# Autodesk Inventor assembly: 2024-210-Angle-Shootaur
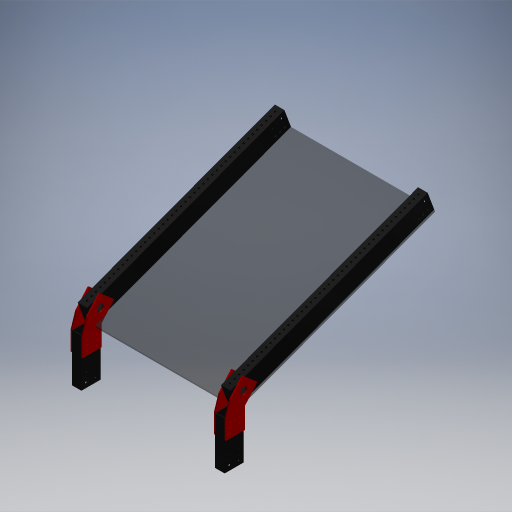
[picture p0: Inventor's stored thumbnail of the model, 512x512]
Saved by Autodesk Inventor 2024.2 (Build 282272000, 272)
## iProperties
Created: 2024-01-23
Part Number: 2024-210-Angle-Shootaur
Document SubType Name: Assembly
Designer: rohan
Author: rohan
## Documents named in this file (5)
- C:\Users\rohan\OneDrive - Hillsborough County Public Schools\Robotics\FIRST-Robotics-Competition\Crescendo\Minotaur-Crescendo-Robot\Structure\Superstructure\Angle-Shootaur\2024-210-Angle-Shootaur.iam
- C:\Users\rohan\OneDrive - Hillsborough County Public Schools\Robotics\FIRST-Robotics-Competition\Crescendo\Minotaur-Crescendo-Robot\Structure\Superstructure\Angle-Shootaur\2024-210-003-Dead-Axle-Gusset.ipt
- C:\Users\rohan\OneDrive - Hillsborough County Public Schools\Robotics\FIRST-Robotics-Competition\Crescendo\Minotaur-Crescendo-Robot\Structure\Superstructure\Angle-Shootaur\2024-210-002-Angle-Beam.ipt
- C:\Users\rohan\OneDrive - Hillsborough County Public Schools\Robotics\FIRST-Robotics-Competition\Crescendo\Minotaur-Crescendo-Robot\Structure\Superstructure\Angle-Shootaur\2024-210-001-Backright-Support.ipt
- C:\Users\rohan\OneDrive - Hillsborough County Public Schools\Robotics\FIRST-Robotics-Competition\Crescendo\Minotaur-Crescendo-Robot\Structure\Superstructure\Polycarbonate-Note-Rest.ipt
## Components (9 placed, 4 different names)
1. 2024-210-003-Dead-Axle-Gusset:1 — Flush:1, Flush:2, Mate:1, Mate:4, Insert:1, Insert:2, Rotational:1
2. 2024-210-003-Dead-Axle-Gusset:2 — Flush:1, Flush:2, Mate:1
3. 2024-210-002-Angle-Beam:1 — Rotational:1, Flush:5, Mate:8, Flush:7, Flush:8
4. 2024-210-001-Backright-Support:1 — Mate:4, Insert:1, Insert:2, Flush:6, Mate:7
5. 2024-210-003-Dead-Axle-Gusset:3
6. 2024-210-003-Dead-Axle-Gusset:4
7. 2024-210-002-Angle-Beam:2 — Flush:5
8. 2024-210-001-Backright-Support:2 — Flush:6, Mate:7
9. Polycarbonate-Note-Rest:1 — Mate:8, Flush:7, Flush:8
## Relationships (20: Flush 8, Mate 6, Insert 4, RevoluteJoint 2)
- Flush:1: 2024-210-003-Dead-Axle-Gusset:1 ↔ 2024-210-003-Dead-Axle-Gusset:2
- Flush:2: 2024-210-003-Dead-Axle-Gusset:1 ↔ 2024-210-003-Dead-Axle-Gusset:2
- Mate:1 (25.4 mm): 2024-210-003-Dead-Axle-Gusset:1 ↔ 2024-210-003-Dead-Axle-Gusset:2
- Mate:4: 2024-210-003-Dead-Axle-Gusset:1 ↔ 2024-210-001-Backright-Support:1
- Insert:1: 2024-210-003-Dead-Axle-Gusset:1 ↔ 2024-210-001-Backright-Support:1
- Insert:2: 2024-210-003-Dead-Axle-Gusset:1 ↔ 2024-210-001-Backright-Support:1
- Rotational:1 [RevoluteJoint] (-3.175 mm): 2024-210-003-Dead-Axle-Gusset:1 ↔ 2024-210-002-Angle-Beam:1
- [Flush]: 2024-210-003-Dead-Axle-Gusset:3 ↔ 2024-210-003-Dead-Axle-Gusset:4
- [Flush]: 2024-210-003-Dead-Axle-Gusset:3 ↔ 2024-210-003-Dead-Axle-Gusset:4
- [Mate] (25.4 mm): 2024-210-003-Dead-Axle-Gusset:3 ↔ 2024-210-003-Dead-Axle-Gusset:4
- [Mate]: 2024-210-003-Dead-Axle-Gusset:3 ↔ 2024-210-001-Backright-Support:2
- [Insert]: 2024-210-003-Dead-Axle-Gusset:3 ↔ 2024-210-001-Backright-Support:2
- [Insert]: 2024-210-003-Dead-Axle-Gusset:3 ↔ 2024-210-001-Backright-Support:2
- [RevoluteJoint] (-3.175 mm): 2024-210-003-Dead-Axle-Gusset:3 ↔ 2024-210-002-Angle-Beam:2
- Flush:5: 2024-210-002-Angle-Beam:1 ↔ 2024-210-002-Angle-Beam:2
- Flush:6: 2024-210-001-Backright-Support:1 ↔ 2024-210-001-Backright-Support:2
- Mate:7 (355.6 mm): 2024-210-001-Backright-Support:1 ↔ 2024-210-001-Backright-Support:2
- Mate:8: 2024-210-002-Angle-Beam:1 ↔ Polycarbonate-Note-Rest:1
- Flush:7: 2024-210-002-Angle-Beam:1 ↔ Polycarbonate-Note-Rest:1
- Flush:8: 2024-210-002-Angle-Beam:1 ↔ Polycarbonate-Note-Rest:1
## Named parameters: d15_d13 = -25 deg, d16_d14 = 0 deg, d17_d2 = 25.4 mm, d18_d5 = 0 mm, d19_d6 = 0 mm, d20_d7 = 0 mm, d21_d10 = -3.175 mm, d22_d11 = -21.901777 deg, d23_d0 = 0 mm, d24_d1 = 0 mm
